# Autodesk Inventor assembly: ProvedoSenzor
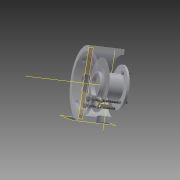
[picture p0: Inventor's stored thumbnail of the model, 180x180]
Saved by Autodesk Inventor 2015 (Build 190159000, 159)
## iProperties
Created: 2014-11-14
Part Number: ProvedoSenzor
Document SubType Name: Assembly
Designer: laca
Author: laca
## Documents named in this file (12)
- C:\Users\laca\Desktop\iRoobo2014Ver3\ProvedoSenzor Tukrozot.iam
- C:\Users\laca\Desktop\iRoobo2014Ver3\BurkolatPVCszenzor.ipt
- C:\Users\laca\Desktop\iRoobo2014Ver3\PorvedoRogzitesAVazhoz.ipt
- C:\Users\laca\Desktop\iRoobo2014Ver3\BurkolatPVCszenzorFedel.ipt
- C:\Users\laca\Desktop\iRoobo2014Ver3\SzenzorSzuportKerek.ipt
- C:\Users\laca\Desktop\iRoobo2014Ver3\InkrementalisOptikaiErzekelo.ipt
- C:\Users\laca\Desktop\iRoobo2014Ver3\InkrementalisFolia.ipt
- C:\Users\laca\Desktop\iRoobo2014Ver3\MerevitesInkrementalisFolia.ipt
- C:\Users\laca\Desktop\iRoobo2014Ver3\Alatet3csavarhoz.ipt
- C:\Users\laca\Desktop\iRoobo2014Ver3\Fi3es40mmcsavar Hexagon.ipt
- C:\Users\laca\Desktop\iRoobo2014Ver3\3asAnya.ipt
- C:\Users\laca\Desktop\iRoobo2014Ver3\KisLemezcsavar.ipt
## Components (23 placed, 11 different names)
1. PorvedoRogzitesAVazhoz:1 — Insert:4, Rotational:28, Rotational:29, Rotational:32, Rotational:33, Flush:3, Rotational:36, Flush:4
2. BurkolatPVCszenzorFedel:1 — Flush:3, Rotational:36, Flush:4
3. SzenzorSzuportKerek:1 — Rigid:1, Insert:2, Insert:3, Insert:4, Mate:1, Insert:5
4. InkrementalisFolia:1 — Rigid:4
5. MerevitesInkrementalisFolia:1 — Rigid:1, Rigid:3, Rigid:4
6. MerevitesInkrementalisFolia:2 — Rigid:3, Flush:5
7. KisLemezcsavar:1 — Insert:2
8. KisLemezcsavar:2 — Insert:3
9. BurkolatPVCszenzor:2
10. InkrementalisOptikaiErzekelo:2 — Cylindrical:5, Cylindrical:6, Rotational:37, Rotational:38, Rotational:39, Rotational:40, Flush:5
11. 3asAnya:2 — Insert:9
12. 3asAnya:4 — Cylindrical:4, Rotational:40
13. 3asAnya:5 — Cylindrical:1, Rotational:39
14. 3asAnya:6 — Insert:8
15. 3asAnya:7 — Cylindrical:3, Rotational:38
16. 3asAnya:8 — Cylindrical:2, Rotational:37
17. Fi3es40mmcsavar Hexagon:3 — Insert:7, Cylindrical:3, Cylindrical:4, Cylindrical:5
18. Fi3es40mmcsavar Hexagon:4 — Insert:6, Cylindrical:1, Cylindrical:2, Cylindrical:6
19. Alatet3csavarhoz:6 — Rotational:29, Insert:7
20. Alatet3csavarhoz:7 — Rotational:28, Insert:9
21. Alatet3csavarhoz:8 — Rotational:33, Insert:6
22. Alatet3csavarhoz:9 — Rotational:32, Insert:8
23. KisLemezcsavar:3 — Insert:5
## Relationships (30: RevoluteJoint 9, Insert 8, CylindricalJoint 6, WeldJoint 3, Flush 3, Mate 1)
- Rigid:1 [WeldJoint] (-8 mm): SzenzorSzuportKerek:1 ↔ MerevitesInkrementalisFolia:1
- Insert:2: SzenzorSzuportKerek:1 ↔ KisLemezcsavar:1
- Insert:3: SzenzorSzuportKerek:1 ↔ KisLemezcsavar:2
- Rigid:3 [WeldJoint]: MerevitesInkrementalisFolia:1 ↔ MerevitesInkrementalisFolia:2
- Insert:4: PorvedoRogzitesAVazhoz:1 ↔ SzenzorSzuportKerek:1
- Mate:1: SzenzorSzuportKerek:1
- Rotational:28 [RevoluteJoint]: PorvedoRogzitesAVazhoz:1 ↔ Alatet3csavarhoz:7
- Rotational:29 [RevoluteJoint]: PorvedoRogzitesAVazhoz:1 ↔ Alatet3csavarhoz:6
- Rotational:32 [RevoluteJoint]: PorvedoRogzitesAVazhoz:1 ↔ Alatet3csavarhoz:9
- Rotational:33 [RevoluteJoint]: PorvedoRogzitesAVazhoz:1 ↔ Alatet3csavarhoz:8
- Flush:3: PorvedoRogzitesAVazhoz:1 ↔ BurkolatPVCszenzorFedel:1
- Rotational:36 [RevoluteJoint]: PorvedoRogzitesAVazhoz:1 ↔ BurkolatPVCszenzorFedel:1
- Flush:4: PorvedoRogzitesAVazhoz:1 ↔ BurkolatPVCszenzorFedel:1
- Insert:5: SzenzorSzuportKerek:1 ↔ KisLemezcsavar:3
- Insert:6: Fi3es40mmcsavar Hexagon:4 ↔ Alatet3csavarhoz:8
- Insert:7: Fi3es40mmcsavar Hexagon:3 ↔ Alatet3csavarhoz:6
- Insert:8: 3asAnya:6 ↔ Alatet3csavarhoz:9
- Insert:9: 3asAnya:2 ↔ Alatet3csavarhoz:7
- Cylindrical:1: 3asAnya:5 ↔ Fi3es40mmcsavar Hexagon:4
- Cylindrical:2: 3asAnya:8 ↔ Fi3es40mmcsavar Hexagon:4
- Cylindrical:3: 3asAnya:7 ↔ Fi3es40mmcsavar Hexagon:3
- Cylindrical:4: 3asAnya:4 ↔ Fi3es40mmcsavar Hexagon:3
- Cylindrical:5: InkrementalisOptikaiErzekelo:2 ↔ Fi3es40mmcsavar Hexagon:3
- Cylindrical:6: InkrementalisOptikaiErzekelo:2 ↔ Fi3es40mmcsavar Hexagon:4
- Rotational:37 [RevoluteJoint]: InkrementalisOptikaiErzekelo:2 ↔ 3asAnya:8
- Rotational:38 [RevoluteJoint]: InkrementalisOptikaiErzekelo:2 ↔ 3asAnya:7
- Rotational:39 [RevoluteJoint]: InkrementalisOptikaiErzekelo:2 ↔ 3asAnya:5
- Rotational:40 [RevoluteJoint]: InkrementalisOptikaiErzekelo:2 ↔ 3asAnya:4
- Flush:5 (-2.5 mm): MerevitesInkrementalisFolia:2 ↔ InkrementalisOptikaiErzekelo:2
- Rigid:4 [WeldJoint]: InkrementalisFolia:1 ↔ MerevitesInkrementalisFolia:1
